# Autodesk Inventor assembly: FingerGeneric
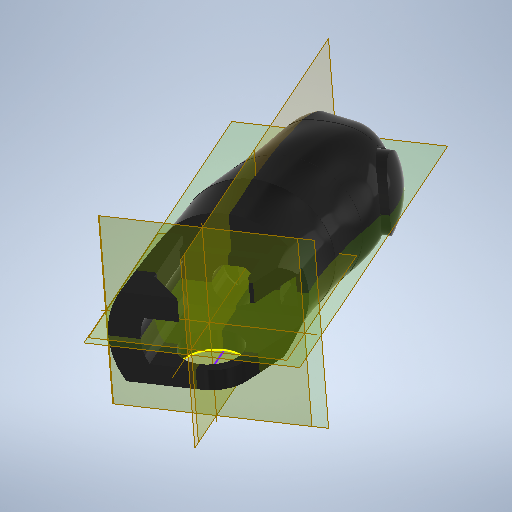
[picture p0: Inventor's stored thumbnail of the model, 512x512]
Saved by Autodesk Inventor 2025.1 (Build 291241000, 241)
## iProperties
Created: 2024-09-11
Part Number: FingerGeneric
Document SubType Name: Assembly
Designer: Alexander
Author: Alexander
## Documents named in this file (6)
- D:\Repositorios_Politecnica\Handi-EPN\CAD\Sim Models\GenericDistalPhalanx.iam
- D:\Repositorios_Politecnica\Handi-EPN\CAD\Right Finger\DP - D Tip.ipt
- D:\Repositorios_Politecnica\Handi-EPN\CAD\Right Finger\DP - D FSR Actuator.ipt
- D:\Repositorios_Politecnica\Handi-EPN\CAD\Right Finger\DP - D Lock.ipt
- D:\Repositorios_Politecnica\Handi-EPN\CAD\Right Finger\DP - D Main.ipt
- D:\Repositorios_Politecnica\Handi-EPN\CAD\Right Finger\DP - P Main R.ipt
## Components (5 placed, 5 different names)
1. DP - D Tip:1 — Mate:3, Flush:5, Mate:4, Mate:6
2. DP - D FSR Actuator:1 — Mate:5, Mate:6, Angle:2
3. DP - D Lock:1 — Mate:1, Mate:2, Angle:1, Mate:7, Flush:6, Flush:7
4. DP - D Main:1 — Mate:3, Flush:5, Mate:4, Mate:5, Mate:7, Flush:6, Flush:7, Angle:2
5. DP - P Main R:1 — Mate:1, Mate:2, Angle:1, Mate:8, Mate:9, Mate:10
## Relationships (15: Mate 10, Flush 3, Angle 2)
- Mate:1: DP - D Lock:1 ↔ DP - P Main R:1
- Mate:2: DP - D Lock:1 ↔ DP - P Main R:1
- Angle:1 (180 deg): DP - D Lock:1 ↔ DP - P Main R:1
- Mate:3: DP - D Tip:1 ↔ DP - D Main:1
- Flush:5: DP - D Tip:1 ↔ DP - D Main:1
- Mate:4: DP - D Tip:1 ↔ DP - D Main:1
- Mate:5: DP - D FSR Actuator:1 ↔ DP - D Main:1
- Mate:6: DP - D Tip:1 ↔ DP - D FSR Actuator:1
- Mate:7: DP - D Lock:1 ↔ DP - D Main:1
- Flush:6: DP - D Lock:1 ↔ DP - D Main:1
- Flush:7: DP - D Lock:1 ↔ DP - D Main:1
- Angle:2 (180 deg): DP - D FSR Actuator:1 ↔ DP - D Main:1
- Mate:8: DP - P Main R:1
- Mate:9: DP - P Main R:1
- Mate:10: DP - P Main R:1
